# Autodesk Inventor assembly: ConnectorBracket
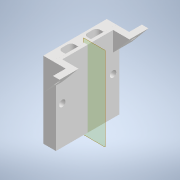
[picture p0: Inventor's stored thumbnail of the model, 180x180]
Saved by Autodesk Inventor 2021 (Build 250183000, 183)
## iProperties
Created: 2022-03-10
Part Number: ConnectorBracket
Document SubType Name: Assembly
Designer: jasmi
Author: jasmi
## Documents named in this file (3)
- D:\2022Robotics\ConnectorBracket.iam
- D:\2022Robotics\conecter bracet cover plate.ipt
- D:\2022Robotics\conecter plate.ipt
## Components (2 placed, 2 different names)
1. conecter bracet cover plate:1 — Flush:1, Mate:1, Flush:2
2. conecter plate:1 — Flush:1, Mate:1, Flush:2
## Relationships (3: Flush 2, Mate 1)
- Flush:1: conecter bracet cover plate:1 ↔ conecter plate:1
- Mate:1: conecter bracet cover plate:1 ↔ conecter plate:1
- Flush:2: conecter bracet cover plate:1 ↔ conecter plate:1
